# Autodesk Inventor assembly: motorisation
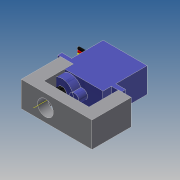
[picture p0: Inventor's stored thumbnail of the model, 180x180]
Saved by Autodesk Inventor 2017 (Build 210142000, 142)
## iProperties
Created: 2018-10-05
Part Number: motorisation
Document SubType Name: Assembly
Designer: Gilles Mottiez
Author: Gilles Mottiez
## Documents named in this file (3)
- C:\Users\Gilles Mottiez\Documents\HES\I5_6\PGA\inventor\motorisation.iam
- C:\Users\Gilles Mottiez\Documents\HES\I5_6\PGA\inventor\support_Servo.ipt
- C:\Users\Gilles Mottiez\Documents\HES\I5_6\PGA\inventor\servo.ipt
## Components (2 placed, 2 different names)
1. support_Servo:1 — Placage:1, Placage:2, Angle:1
2. servo:1 — Placage:1, Placage:2, Angle:1
## Relationships (3: Mate 2, Angle 1)
- Placage:1 [Mate]: support_Servo:1 ↔ servo:1
- Placage:2 [Mate]: support_Servo:1 ↔ servo:1
- Angle:1 (0 deg): support_Servo:1 ↔ servo:1
